# Autodesk Inventor assembly: general
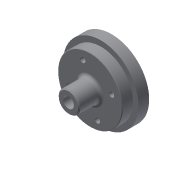
[picture p0: Inventor's stored thumbnail of the model, 180x180]
Saved by Autodesk Inventor 2022 (Build 260148000, 148)
## iProperties
Created: 2006-05-26
Part Number: general
Document SubType Name: Assembly
Designer: Administrator
Author: Administrator
## Documents named in this file (3)
- C:\Autodesk Inventor 2022 Advanced Assembly Modeling Practice Files\Design_Accelerator2\general.iam
- C:\Autodesk Inventor 2022 Advanced Assembly Modeling Practice Files\Design_Accelerator2\plate.ipt
- C:\Autodesk Inventor 2022 Advanced Assembly Modeling Practice Files\Design_Accelerator2\flange.ipt
## Components (2 placed, 2 different names)
1. flange:1 — Mate:1, Mate:2
2. plate:1 — Mate:1, Mate:2
## Relationships (2: Mate 2)
- Mate:1: flange:1 ↔ plate:1
- Mate:2: flange:1 ↔ plate:1
